# Autodesk Inventor assembly: ExplodedView_CameraMount
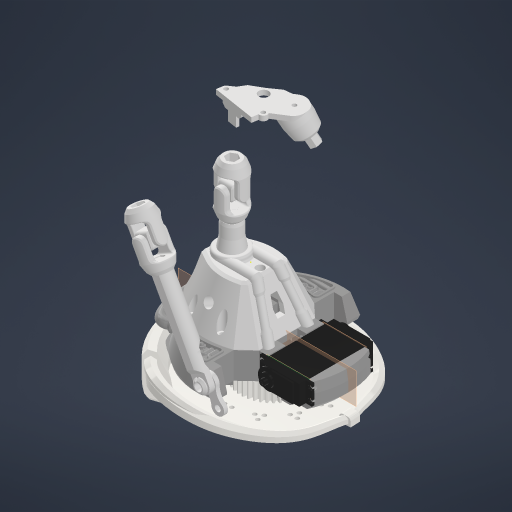
[picture p0: Inventor's stored thumbnail of the model, 512x512]
Saved by Autodesk Inventor 2024 (Build 280153000, 153)
## iProperties
Created: 2025-09-16
Part Number: ExplodedView_CameraMount
Document SubType Name: Assembly
Designer: kevin
Author: kevin
## Documents named in this file (10)
- C:\Users\kevin\Desktop\SeniorDesign\ExplodedView_CameraMount.iam
- C:\Users\kevin\Desktop\Camera_Baseplate.ipt
- C:\Users\kevin\Desktop\SeniorDesign\MG996R.ipt
- C:\Users\kevin\Desktop\SeniorDesign\Gear_Cover.ipt
- C:\Users\kevin\Desktop\SeniorDesign\Servo_Shaft.iam
- C:\Users\kevin\Desktop\SeniorDesign\Universal_Joint.iam
- C:\Users\kevin\Desktop\Neck_Cover.ipt
- C:\Users\kevin\Desktop\Camera_Mount\Design Accelerator\Spur Gears2.iam
- C:\Users\kevin\Desktop\Camera_Mount\Design Accelerator\Spur Gear11.ipt
- C:\Users\kevin\Desktop\SeniorDesign\Head_Baseplate_Legacy.ipt
## Components (12 placed, 9 different names)
1. Camera_Baseplate:1 — Mate:1, Mate:2, Mate:3, Mate:4, Mate:5, Mate:6, Mate:7, Mate:9, Mate:10, Mate:13, Mate:14, Mate:21, Mate:24, Mate:25, Mate:26
2. MG996R:1 — Mate:1, Mate:3, Mate:6, Mate:11
3. MG996R:2 — Mate:2, Mate:4, Mate:5
4. MG996R:3 — Mate:7, Mate:9, Mate:10, Mate:22, Mate:23
5. Gear_Cover:1 — Mate:24
6. Servo_Shaft:1 [sub-assembly] — Mate:11, Mate:17, Mate:18
7. Universal_Joint:1 [sub-assembly] — Mate:15, Mate:16, Mate:27
8. Universal_Joint:3 [sub-assembly] — Mate:17, Mate:18
9. Neck_Cover:1 — Mate:13, Mate:14, Mate:15, Mate:16, Mate:26
10. Spur Gears:1 [sub-assembly] — Mate:21, Mate:25
11. Spur Gear1:1 — Mate:22, Mate:23
12. Head_Baseplate_Legacy:1 — Mate:27
## Relationships (23: Mate 23)
- Mate:1: Camera_Baseplate:1 ↔ MG996R:1
- Mate:2: Camera_Baseplate:1 ↔ MG996R:2
- Mate:3: Camera_Baseplate:1 ↔ MG996R:1
- Mate:4: Camera_Baseplate:1 ↔ MG996R:2
- Mate:5 (0.5 mm): Camera_Baseplate:1 ↔ MG996R:2
- Mate:6 (0.5 mm): Camera_Baseplate:1 ↔ MG996R:1
- Mate:7: Camera_Baseplate:1 ↔ MG996R:3
- Mate:9: Camera_Baseplate:1 ↔ MG996R:3
- Mate:10: Camera_Baseplate:1 ↔ MG996R:3
- Mate:11: MG996R:1 ↔ Servo_Shaft:1
- Mate:13: Camera_Baseplate:1 ↔ Neck_Cover:1
- Mate:14: Camera_Baseplate:1 ↔ Neck_Cover:1
- Mate:15: Universal_Joint:1 ↔ Neck_Cover:1
- Mate:16: Universal_Joint:1 ↔ Neck_Cover:1
- Mate:17: Servo_Shaft:1 ↔ Universal_Joint:3
- Mate:18: Servo_Shaft:1 ↔ Universal_Joint:3
- Mate:21: Camera_Baseplate:1 ↔ Spur Gears:1
- Mate:22: MG996R:3 ↔ Spur Gear1:1
- Mate:23: MG996R:3 ↔ Spur Gear1:1
- Mate:24: Camera_Baseplate:1 ↔ Gear_Cover:1
- Mate:25: Camera_Baseplate:1 ↔ Spur Gears:1
- Mate:26: Camera_Baseplate:1 ↔ Neck_Cover:1
- Mate:27: Universal_Joint:1 ↔ Head_Baseplate_Legacy:1
